# Autodesk Inventor assembly: CaseAssemblyv3
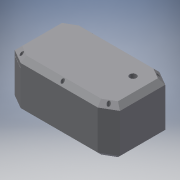
[picture p0: Inventor's stored thumbnail of the model, 180x180]
Saved by Autodesk Inventor 2017 (Build 210142000, 142)
## iProperties
Created: 2020-03-12
Part Number: CaseAssemblyv3
Document SubType Name: Assembly
Designer: Manny
Author: Manny
## Documents named in this file (4)
- C:\Users\Owner\Documents\ENG Year 5\Capstone\CaseAssemblyv3.iam
- C:\Users\Owner\Documents\ENG Year 5\Capstone\Bottomv3.ipt
- C:\Users\Owner\Documents\ENG Year 5\Capstone\Topv3.ipt
- C:\Users\Owner\Documents\ENG Year 5\Capstone\BatteryCover.ipt
## Components (3 placed, 3 different names)
1. Bottomv3:1 — Mate:1, Flush:1, Flush:2, Mate:2, Mate:3, Mate:4
2. Topv3:1 — Mate:1, Flush:1, Flush:2
3. BatteryCover:1 — Mate:2, Mate:3, Mate:4
## Relationships (6: Mate 4, Flush 2)
- Mate:1: Bottomv3:1 ↔ Topv3:1
- Flush:1: Bottomv3:1 ↔ Topv3:1
- Flush:2: Bottomv3:1 ↔ Topv3:1
- Mate:2: Bottomv3:1 ↔ BatteryCover:1
- Mate:3: Bottomv3:1 ↔ BatteryCover:1
- Mate:4: Bottomv3:1 ↔ BatteryCover:1
